# Autodesk Inventor assembly: 00_XY_stage-CHUO_SEIKI_LD-647-R1
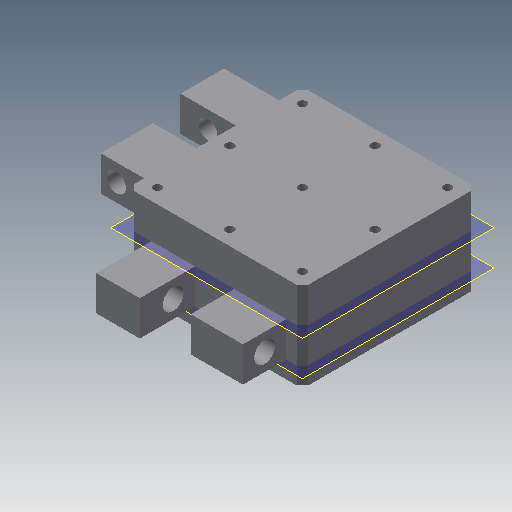
[picture p0: Inventor's stored thumbnail of the model, 512x512]
Saved by Autodesk Inventor 2019 (Build 230136000, 136)
## iProperties
Created: 2019-05-02
Part Number: 00_XY_stage-CHUO_SEIKI_LD-647-R1
Document SubType Name: Assembly
Designer: diederichbenedict
Author: diederichbenedict
## Documents named in this file (4)
- C:\Users\diederichbenedict\Dropbox\Dokumente\Promotion\PROJECTS\STORMoChip\GITHUB\CAD\Nanoscopy-on-the-cheap\Workspace\00_XY_stage-Chinese_60x60.iam
- C:\Users\diederichbenedict\Dropbox\Dokumente\Promotion\PROJECTS\STORMoChip\GITHUB\CAD\Nanoscopy-on-the-cheap\Workspace\00_XY_stage-Chinese_60x60-Top.ipt
- C:\Users\diederichbenedict\Dropbox\Dokumente\Promotion\PROJECTS\STORMoChip\GITHUB\CAD\Nanoscopy-on-the-cheap\Workspace\00_XY_stage-Chinese_60x60-Middle.ipt
- C:\Users\diederichbenedict\Dropbox\Dokumente\Promotion\PROJECTS\STORMoChip\GITHUB\CAD\Nanoscopy-on-the-cheap\Workspace\00_XY_stage-Chinese_60x60-Bottom.ipt
## Components (3 placed, 3 different names)
1. 00_XY_stage-Chinese_60x60-Top:1 — Flush:1, Flush:2
2. 00_XY_stage-Chinese_60x60-Middle:1 — Flush:1, Flush:2, Flush:3, Flush:4
3. 00_XY_stage-Chinese_60x60-Bottom:1 — Flush:3, Flush:4
## Relationships (4: Flush 4)
- Flush:1: 00_XY_stage-Chinese_60x60-Top:1 ↔ 00_XY_stage-Chinese_60x60-Middle:1
- Flush:2: 00_XY_stage-Chinese_60x60-Top:1 ↔ 00_XY_stage-Chinese_60x60-Middle:1
- Flush:3: 00_XY_stage-Chinese_60x60-Middle:1 ↔ 00_XY_stage-Chinese_60x60-Bottom:1
- Flush:4: 00_XY_stage-Chinese_60x60-Middle:1 ↔ 00_XY_stage-Chinese_60x60-Bottom:1
